(part 1 of 3)
# Autodesk Inventor assembly: FinalAssembly
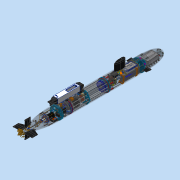
[picture p0: Inventor's stored thumbnail of the model, 180x180]
Saved by Autodesk Inventor 2018 (Build 220112000, 112)
## iProperties
Created: 2016-12-11
Part Number: FinalAssembly
Document SubType Name: Assembly
Designer: techn
Mass: 4957.63 g
Surface Area: 18369.4 cm^2
Volume: 2887.61 cm^3
Density: 1.71686 g/cm^3
Author: techn
## Documents named in this file (168)
- D:\Projects\Submarine-project\CAD\FinalAssembly.iam
- D:\Projects\Submarine-project\CAD\aft\AftSectionAirtightRear.ipt
- D:\Projects\Submarine-project\CAD\aft\AftSectionWithSteeringLinkages.ipt
- D:\Projects\Submarine-project\CAD\aft\RearmostAftSection.ipt
- D:\Projects\Submarine-project\CAD\common\steeringYoke3mmShaft.ipt
- D:\Projects\Submarine-project\CAD\aft\aftSectionAirtightCap.ipt
- D:\Projects\Submarine-project\CAD\common\AluminumSealingDisc.ipt
- D:\Projects\Submarine-project\CAD\midships\AftServoSection\rearServoAttachmentPlate.ipt
- D:\Projects\Submarine-project\CAD\common\HitecServo\HitecServoAssembly.iam
- D:\Projects\Submarine-project\CAD\common\HitecServo\ServoHorn10mmPitch.ipt
- D:\Projects\Submarine-project\CAD\aft\planeLinkages\2mmBentFromSealDive.ipt
- D:\Projects\Submarine-project\CAD\aft\planeLinkages\2mmToDive.ipt
- D:\Projects\Submarine-project\CAD\aft\planeLinkages\2mmToSeal.ipt
- D:\Projects\Submarine-project\CAD\aft\planeLinkages\2mmToServo.ipt
- D:\Projects\Submarine-project\CAD\aft\planeLinkages\metalClevisis.ipt
- D:\Projects\Submarine-project\CAD\aft\planeLinkages\2mmBentFromSealRudder.ipt
- D:\Projects\Submarine-project\CAD\aft\planeLinkages\2mmToRudder.ipt
- D:\Projects\Submarine-project\CAD\common\screws\flatPlasticScrewSmall.ipt
- D:\Projects\Submarine-project\CAD\common\YokeDowelPins.ipt
- D:\Projects\Submarine-project\CAD\aft\RudderStabilizingLowerFins.ipt
- D:\Projects\Submarine-project\CAD\common\SleeveBearing3mmFlanged.ipt
- D:\Projects\Submarine-project\CAD\aft\DivePlanesStabilizingFins.ipt
- D:\Projects\Submarine-project\CAD\aft\RudderStabilizingFinBottom.ipt
- D:\Projects\Submarine-project\CAD\aft\RudderStabilizingFins.ipt
- D:\Projects\Submarine-project\CAD\aft\3mmControlSurfaceShaft_1.ipt
- D:\Projects\Submarine-project\CAD\aft\3mmControlSurfaceShaft_2.ipt
- D:\Projects\Submarine-project\CAD\aft\DivePlanesControlSurface.ipt
- D:\Projects\Submarine-project\CAD\aft\RudderLowerControlSurface.ipt
- D:\Projects\Submarine-project\CAD\aft\RudderUpperControlSurface.ipt
- D:\Projects\Submarine-project\CAD\common\screws\ScrewPlastic_4_20_.625inch.ipt
- D:\Projects\Submarine-project\CAD\common\ThreadedRod_Nuts_Bolts\NarrowHexNutThread_5_40.ipt
- D:\Projects\Submarine-project\CAD\common\ORingA50_.25OD_.125ID.ipt
- D:\Projects\Submarine-project\CAD\common\ThreadedRod_Nuts_Bolts\Bolt_ButtonHead_Hex_Thread_5_40_1inch.ipt
- D:\Projects\Submarine-project\CAD\aft\MotorAssembly0.iam
- D:\Projects\Submarine-project\CAD\common\PushRodSeal\Engel3mm\Engel3mmAssembly.iam
- D:\Projects\Submarine-project\CAD\common\ThreadedRod_Nuts_Bolts\Bolt_Buttonhead_Hex_Thread_5_40_.625inch.ipt
- D:\Projects\Submarine-project\CAD\common\ORingA50_1.296ID_1.574OD.ipt
- D:\Projects\Submarine-project\CAD\midships\ElectronicsSection\QUICRUN ESC\QuicrunESCAssembly.iam
- D:\Projects\Submarine-project\CAD\common\screws\ScrewPlastic_4_20_.75inch_Flat.ipt
- D:\Projects\Submarine-project\CAD\common\ThreadedRod_Nuts_Bolts\Bolt_FlatHead_Hex_Thread_M3_8mm.ipt
- D:\Projects\Submarine-project\CAD\common\ORingA50_3.75OD_3.5ID_Compressed.ipt
- D:\Projects\Submarine-project\CAD\midships\AftServoSection\frontServoAttachmentPlate.ipt
- D:\Projects\Submarine-project\CAD\midships\AluminumSealingDiscMidshipsRear.ipt
- D:\Projects\Submarine-project\CAD\midships\SpoolSection\aftSpoolSectionSealingWall.ipt
- D:\Projects\Submarine-project\CAD\common\3mmShaftToServo\ServoWithShaftAssembly.iam
- D:\Projects\Submarine-project\CAD\common\screws\ScrewPlastic_4_20_.5inch.ipt
- D:\Projects\Submarine-project\CAD\common\ORingA70_.176ID_.316OD.ipt
- D:\Projects\Submarine-project\CAD\midships\ElectronicsSection\aluminumWiringTubing.ipt
- D:\Projects\Submarine-project\CAD\common\ThreadedRod_Nuts_Bolts\aftThreadedRodThread_5_40.ipt
- D:\Projects\Submarine-project\CAD\common\SleeveBearing.125inch.ipt
- D:\Projects\Submarine-project\CAD\common\BallBearing4mmFlanged.ipt
- D:\Projects\Submarine-project\CAD\midships\BallastSection\bearing_1_8inch.ipt
- D:\Projects\Submarine-project\CAD\midships\SpoolSection\PinionGear.ipt
- D:\Projects\Submarine-project\CAD\midships\SpoolSection\SpoolAxle.ipt
- D:\Projects\Submarine-project\CAD\midships\BallastSection\smallIdlerPinion.ipt
- D:\Projects\Submarine-project\CAD\midships\SpoolSection\SpoolSectionSealingWallFront.ipt
- D:\Projects\Submarine-project\CAD\midships\SpoolSection\FixedCylinderWireStorage.ipt
- D:\Projects\Submarine-project\CAD\midships\SpoolSection\FixedCylinderWireStorageInsert.ipt
- D:\Projects\Submarine-project\CAD\midships\BallastSection\pistonTank.ipt
- D:\Projects\Submarine-project\CAD\common\SleeveBearing3mm.ipt
- D:\Projects\Submarine-project\CAD\midships\BallastSection\pistonSealingWallFront.ipt
- D:\Projects\Submarine-project\CAD\midships\BallastSection\pistonSealingDisc.ipt
- D:\Projects\Submarine-project\CAD\midships\BallastSection\pistonSealingWallRear.ipt
- D:\Projects\Submarine-project\CAD\common\ThreadedRod_Nuts_Bolts\WeldNutThread_5_16_18.ipt
- D:\Projects\Submarine-project\CAD\common\ThreadedRod_Nuts_Bolts\ThreadedRodThread_5_16_18.ipt
- D:\Projects\Submarine-project\CAD\common\ThreadedRod_Nuts_Bolts\HexNutThread_5_16_18.ipt
- D:\Projects\Submarine-project\CAD\common\ThreadedRod_Nuts_Bolts\WasherForThread_5_16_18.ipt
- D:\Projects\Submarine-project\CAD\midships\BallastSection\forwardBallastSealingWallRear.ipt
- D:\Projects\Submarine-project\CAD\midships\BallastSection\forwardBallastSealingWallFront.ipt
- D:\Projects\Submarine-project\CAD\midships\BallastSection\forwardBallastSealingWallDisc.ipt
- D:\Projects\Submarine-project\CAD\common\ThreadedRod_Nuts_Bolts\midshipsThreadedRodThread_5_40.ipt
- D:\Projects\Submarine-project\CAD\midships\BallastSection\pushSwitchBushingHolder.ipt
- D:\Projects\Submarine-project\CAD\midships\BallastSection\pushSwitchRod.ipt
- D:\Projects\Submarine-project\CAD\midships\BallastSection\pushSwitchSpring.ipt
- D:\Projects\Submarine-project\CAD\midships\BallastSection\RadialBearingMountCover.ipt
- D:\Projects\Submarine-project\CAD\midships\BallastSection\ThrustWasher.ipt
- D:\Projects\Submarine-project\CAD\midships\BallastSection\pistonSpurGear.ipt
- D:\Projects\Submarine-project\CAD\midships\BallastSection\retentionStandoffs.ipt
- D:\Projects\Submarine-project\CAD\midships\BallastSection\SpurGearThrustDistributer.ipt
- D:\Projects\Submarine-project\CAD\midships\BallastSection\ThrustBearingMount.ipt
- D:\Projects\Submarine-project\CAD\midships\BallastSection\idlerShaftBearingMount.ipt
- D:\Projects\Submarine-project\CAD\aft\540DCMotor.ipt
- D:\Projects\Submarine-project\CAD\midships\BallastSection\limitSwitchPushHolder1.ipt
- D:\Projects\Submarine-project\CAD\common\ThreadedRod_Nuts_Bolts\WeldNutThread_5_16_18_Cut.ipt
- D:\Projects\Submarine-project\CAD\midships\BallastSection\limitSwitchHolder2Backplate.ipt
- D:\Projects\Submarine-project\CAD\common\Switches\LimitSwitch\LIMIT SWITCH.ipt
- D:\Projects\Submarine-project\CAD\midships\BallastSection\limitSwitchHolderMount.ipt
- D:\Projects\Submarine-project\CAD\midships\BallastSection\limitSwitchHolder2.ipt
- D:\Projects\Submarine-project\CAD\common\Switches\LimitSwitch\LimitSwitchAssembly.iam
- D:\Projects\Submarine-project\CAD\midships\BallastSection\idlerShaft.ipt
- D:\Projects\Submarine-project\CAD\midships\BallastSection\largeIdlerPinion.ipt
- D:\Projects\Submarine-project\CAD\midships\BallastSection\BearingRetentionBrace.ipt
- D:\Projects\Submarine-project\CAD\midships\ElectronicsSection\foreElectronicsSealingWallRear.ipt
- D:\Projects\Submarine-project\CAD\midships\ElectronicsSection\foreElectronicsSealingDisc.ipt
- D:\Projects\Submarine-project\CAD\midships\ElectronicsSection\foreElectronicsSealingWallFront.ipt
- D:\Projects\Submarine-project\CAD\midships\ElectronicsSection\foreElectronicsSealingWallFrontCap.ipt
- D:\Projects\Submarine-project\CAD\midships\3mmControlSurfaceShaftForePlanes.ipt
- D:\Projects\Submarine-project\CAD\midships\foreDivePlanes.ipt
- D:\Projects\Submarine-project\CAD\midships\foreDivePlanesLinkage.ipt
- D:\Projects\Submarine-project\CAD\fore\foreHullLower.ipt
- D:\Projects\Submarine-project\CAD\fore\foreHullInsert.ipt
- D:\Projects\Submarine-project\CAD\fore\foreHullUpper.ipt
- D:\Projects\Submarine-project\CAD\midships\ElectronicsSection\ArduinoMegaHolder1.ipt
- D:\Projects\Submarine-project\CAD\midships\ElectronicsSection\ArduinoMegaHolder2.ipt
- D:\Projects\Submarine-project\CAD\midships\ElectronicsSection\ArduinoMega.ipt
- D:\Projects\Submarine-project\CAD\midships\ElectronicsSection\ServoControllerHolder.ipt
- D:\Projects\Submarine-project\CAD\midships\ElectronicsSection\ServoController\ServoControllerAssembly.iam
- D:\Projects\Submarine-project\CAD\midships\ElectronicsSection\ArduinoNanoHolder.ipt
- D:\Projects\Submarine-project\CAD\midships\ElectronicsSection\ArduinoNanoHolderSide2.ipt
- D:\Projects\Submarine-project\CAD\midships\ElectronicsSection\ArduinoNanoNoPins.iam
- D:\Projects\Submarine-project\CAD\midships\ElectronicsSection\BEC\BEC_Assembly.iam
- D:\Projects\Submarine-project\CAD\midships\PrimaryHullLexanTube_01.ipt
- D:\Projects\Submarine-project\CAD\common\5mmLED.ipt
- D:\Projects\Submarine-project\CAD\ASDS\ASDSAssembly.iam
- D:\Projects\Submarine-project\CAD\common\DriveBattery.ipt
- D:\Projects\Submarine-project\CAD\common\DriveBatteryHolder.ipt
- D:\Projects\Submarine-project\CAD\common\ElectronicsBatteryAssembly.iam
- D:\Projects\Submarine-project\CAD\common\PressureSensor.ipt
- D:\Projects\Submarine-project\CAD\midships\Sail\SailAssembly\SailAssembly.iam
- D:\Projects\Submarine-project\CAD\midships\ElectronicsSection\BackupNanoCase.iam
- D:\Projects\Submarine-project\CAD\common\RelayModule.ipt
- D:\Projects\Submarine-project\CAD\midships\Sail\WireGuide.ipt
- D:\Projects\Submarine-project\CAD\midships\Sail\WireGuideToSail1.ipt
- D:\Projects\Submarine-project\CAD\midships\Sail\WireGuideToSail2.ipt
- D:\Projects\Submarine-project\CAD\midships\Sail\WireGuideToMiniSub.ipt
- D:\Projects\Submarine-project\CAD\midships\Sail\WireGuideToMiniSubExtender.ipt
- D:\Projects\Submarine-project\CAD\midships\SpoolSection\SmallSpoolAssembly.iam
- D:\Projects\Submarine-project\CAD\midships\SpoolSection\CarriageImproved.ipt
- D:\Projects\Submarine-project\CAD\midships\AftServoSection\MiniSpoolServoShaft.ipt
- D:\Projects\Submarine-project\CAD\midships\AftServoSection\CarriageConnectorShaft.ipt
- D:\Projects\Submarine-project\CAD\midships\SpoolSection\carriageRideShaft.ipt
- D:\Projects\Submarine-project\CAD\common\ThreadedRod_Nuts_Bolts\spoolCarriageThreadedRodThread_5_40.ipt
- D:\Projects\Submarine-project\CAD\common\ThreadedRod_Nuts_Bolts\aftServoSectionThreadedRodThread_5_40.ipt
- D:\Projects\Submarine-project\CAD\common\PinionGear20T.ipt
- D:\Projects\Submarine-project\CAD\midships\SpoolSection\CarrageRodEndMount.ipt
- D:\Projects\Submarine-project\CAD\midships\AftServoSection\SpoolServoMount.ipt
- D:\Projects\Submarine-project\CAD\common\ORingA70_2.484ID_2.762OD_Compressed.ipt
- D:\Projects\Submarine-project\CAD\common\NarrowHexNutCaps.ipt
- D:\Projects\Submarine-project\CAD\aft\encoder\4mmShaftCollar.ipt
- D:\Projects\Submarine-project\CAD\aft\encoder\ShaftCollarMagnetMount.ipt
- D:\Projects\Submarine-project\CAD\aft\encoder\EncoderMagnet.ipt
- D:\Projects\Submarine-project\CAD\midships\BallastSection\idlerShaft2.ipt
- D:\Projects\Submarine-project\CAD\common\ThreadedRod_Nuts_Bolts\Bolt_SocketHead_Hex_Thread_M3_16mm.ipt
- D:\Projects\Submarine-project\CAD\midships\BallastSection\CompressionWasherPlastic.ipt
- D:\Projects\Submarine-project\CAD\common\ThreadedRod_Nuts_Bolts\HexNutThread_M3.ipt
- D:\Projects\Submarine-project\CAD\midships\BallastSection\ThrustWasherPrimary.ipt
- D:\Projects\Submarine-project\CAD\midships\BallastSection\pushSwitchRodSpacer.ipt
- D:\Projects\Submarine-project\CAD\midships\BallastSection\RadialBearingLarge.ipt
- D:\Projects\Submarine-project\CAD\Downloaded\ScimitarProp\ScimitarPropellerModel1.iam
- D:\Projects\Submarine-project\CAD\common\MicroGearMotor\MicroGearMotor.ipt
- D:\Projects\Submarine-project\CAD\common\3mm_.125inch_ShaftCoupler.ipt
- D:\Projects\Submarine-project\CAD\common\MicroGearMotor\GearMotorMount.ipt
- D:\Projects\Submarine-project\CAD\midships\ASDSAttachment\ASDSAttachmentAssemblyUpdated.iam
- D:\Projects\Submarine-project\CAD\midships\ASDSAttachment\RearMount.ipt
- D:\Projects\Submarine-project\CAD\aft\encoder\hallEffectSensorAssembly.iam
- D:\Projects\Submarine-project\CAD\midships\BallastSection\gearboxBearingHolderForward.ipt
- D:\Projects\Submarine-project\CAD\midships\BallastSection\gearboxBearingHolderHexNutBacking.ipt
- D:\Projects\Submarine-project\CAD\common\ThreadedRod_Nuts_Bolts\Bolt_SocketHead_Hex_Thread_M3_8mm.ipt
- D:\Projects\Submarine-project\CAD\common\ThreadedRod_Nuts_Bolts\Bolt_ButtonHead_Hex_Thread_M3_10mm.ipt
- D:\Projects\Submarine-project\CAD\common\MicroGearMotor\GearMotorMountArm.ipt
- D:\Projects\Submarine-project\CAD\midships\AftServoSection\HallEffectSpoolSensorMount2.ipt
- D:\Projects\Submarine-project\CAD\aft\encoder\HallEffectSensor.ipt
- D:\Projects\Submarine-project\CAD\midships\AftServoSection\SpoolCarrageMagnetMountREV2.ipt
- D:\Projects\Submarine-project\CAD\midships\AftServoSection\HallEffectSpoolSensorMount3.ipt
- D:\Projects\Submarine-project\CAD\midships\AftServoSection\HallEffectSpoolSensorMount3Brace.ipt
- D:\Projects\Submarine-project\CAD\midships\BallastSection\HallEffectSpoolSensorMount3.ipt
- D:\Projects\Submarine-project\CAD\midships\ElectronicsSection\RelayHolderREV2.ipt
- D:\Projects\Submarine-project\CAD\SlipRing\SlipRingAssy.iam
## Components (560 placed, 166 different names)
1. AftSectionAirtightRear:1 — Mate:1, Mate:5, Mate:6, Mate:101, Mate:205, Angle:13, Mate:221, Mate:223, Mate:224, Mate:225, Angle:15, Mate:226, Mate:227, Angle:16, Rigid:11, Mate:228, Mate:229, Rigid:12, Flush:16, Flush:54, Flush:55, Mate:428, Mate:436, Mate:437, Mate:441, Mate:700
2. AftSectionWithSteeringLinkages:1 — Mate:1, Mate:30, Mate:31, Mate:190, Angle:11, Mate:436, Mate:1031, Rigid:38, Rigid:39, Mate:1061, Mate:1062, Mate:1063, Mate:1064, Mate:1065
3. AluminumSealingDisc:1 — Mate:8, Mate:10, Mate:11, Mate:12, Mate:13, Mate:102, Rigid:13
4. rearServoAttachmentPlate:1 — Mate:11, Mate:12, Mate:13, Mate:14, Mate:16, Mate:17, Mate:18, Mate:19, Mate:249, Mate:261, Mate:275, Mate:427, Mate:858
5. HitecServoAssembly:1 [sub-assembly] — Mate:14, Mate:16, Mate:20, Mate:23, Angle:5, Flush:17, Mate:293, Mate:296, Mate:297, Angle:26, Mate:427, Angle:82
6. HitecServoAssembly:2 [sub-assembly] — Mate:17, Mate:18, Mate:19, Mate:21, Mate:22, Angle:4, Angle:18, Angle:70, Angle:84
7. ServoHorn10mmPitch:1 — Mate:20, Mate:23, Mate:37, Angle:5
8. ServoHorn10mmPitch:2 — Mate:21, Mate:22, Mate:36, Angle:4
9. aftSectionAirtightCap:2 — Mate:5, Mate:6, Mate:8, Mate:10, Mate:101, Mate:102, Mate:219, Mate:220, Angle:14, Mate:244, Flush:18, Mate:701
10. RearmostAftSection:2 — Mate:28, Mate:29, Mate:30, Mate:31, Mate:109, Mate:110, Mate:111, Mate:112, Mate:113, Mate:114, Mate:118, Mate:119, Mate:120, Mate:121, Mate:122, Mate:123, Mate:124, Mate:125, Mate:126, Mate:127, Mate:128, Mate:129, Mate:130, Mate:131, Mate:132, Mate:133, Mate:134, Mate:135, Mate:136, Angle:6, Mate:137, Mate:138, Angle:7, Mate:160, Mate:161, Mate:162, Mate:163, Mate:164, Mate:165, Mate:166, Mate:167, Mate:168, Mate:169, Mate:170, Mate:171, Mate:206, Mate:216, Mate:313, Mate:314, Mate:438, Mate:439, Mate:440
11. BallBearing4mmFlanged:1 — Mate:313, Mate:314, Mate:1030
12. steeringYoke3mmShaft:3 — Mate:29, Mate:59, Mate:60, Flush:8, Flush:9, Rigid:1
13. steeringYoke3mmShaft:4 — Mate:28, Mate:61, Mate:77, Rigid:2
14. metalClevisis:5 — Mate:36, Mate:71, Mate:72, Mate:707, Flush:113
15. metalClevisis:6 — Mate:37, Mate:55, Mate:56, Mate:706, Flush:112
16. 2mmToServo:7 — Mate:55, Mate:56, Ball:3
17. 2mmToSeal:4 — Ball:2
18. 2mmToSeal:5 — Ball:3
19. 2mmToDive:1 — Ball:1
20. metalClevisis:7 — Mate:59, Mate:60, Mate:69, Mate:70, Flush:7, Mate:430
21. metalClevisis:8 — Mate:61, Mate:75, Mate:76, Mate:77, Flush:6, Mate:429
22. 2mmBentFromSealDive:2 — Ball:1, Mate:69, Mate:70
23. 2mmToServo:8 — Ball:2, Mate:71, Mate:72
24. 2mmToRudder:1 — Ball:4
25. 2mmBentFromSealRudder:2 — Ball:4, Mate:75, Mate:76
26. YokeDowelPins:1 — Flush:6, Mate:429
27. YokeDowelPins:2 — Flush:7, Mate:430
28. RudderStabilizingLowerFins:1 — Mate:109, Mate:110, Mate:111
29. RudderStabilizingLowerFins:2 — Mate:112, Mate:113, Mate:114, Mate:158
30. RudderStabilizingLowerFins:3 — Mate:438, Mate:439, Mate:440
31. RudderStabilizingLowerFins:4 — Mate:118, Mate:119, Mate:120
32. SleeveBearing3mmFlanged:1 — Mate:121, Mate:122, Mate:141
33. SleeveBearing3mmFlanged:2 — Mate:127, Mate:128, Mate:139
34. SleeveBearing3mmFlanged:3 — Mate:125, Mate:126, Mate:142
35. SleeveBearing3mmFlanged:4 — Mate:123, Mate:124, Mate:140
36. DivePlanesStabilizingFins:1 — Mate:129, Mate:133, Mate:134
37. DivePlanesStabilizingFins:2 — Mate:130, Mate:131, Mate:132, Mate:148
38. RudderStabilizingFinBottom:1 — Mate:137, Mate:138, Angle:7
39. RudderStabilizingFins:1 — Mate:135, Mate:136, Angle:6
40. 3mmControlSurfaceShaft_1:1 — Mate:139, Mate:143, Mate:144, Flush:9, Rigid:1
41. 3mmControlSurfaceShaft_1:2 — Mate:140, Mate:147, Mate:150, Flush:8
42. 3mmControlSurfaceShaft_2:1 — Mate:141, Mate:153, Mate:154, Rigid:2
43. 3mmControlSurfaceShaft_2:2 — Mate:142, Mate:155, Mate:156
44. DivePlanesControlSurface:1 — Mate:143, Mate:144, Mate:149
45. DivePlanesControlSurface:2 — Mate:147, Mate:148, Mate:149, Mate:150
46. YokeDowelPins:3 — Mate:707, Flush:113
47. YokeDowelPins:4 — Mate:706, Flush:112
48. RudderLowerControlSurface:1 — Mate:155, Mate:156, Mate:158, Mate:159
49. RudderUpperControlSurface:1 — Mate:153, Mate:154, Mate:159
50. ScrewPlastic_4_20_.625inch:1 — Mate:160, Mate:161
51. ScrewPlastic_4_20_.625inch:2 — Mate:162, Mate:163
52. ScrewPlastic_4_20_.625inch:3 — Mate:166, Mate:167
53. ScrewPlastic_4_20_.625inch:6 — Mate:170, Mate:171
54. ScrewPlastic_4_20_.625inch:7 — Mate:164, Mate:165
55. ScrewPlastic_4_20_.625inch:8 — Mate:168, Mate:169
56. MotorAssembly0:1 [sub-assembly] — Mate:221, Mate:223, Mate:231, Tangent:1, Mate:259, Mate:260, Flush:20, Flush:21, Mate:441, Mate:921, Mate:1029
57. Engel3mmAssembly:1 [sub-assembly] — Mate:226, Mate:227, Angle:16, Angle:17
58. Engel3mmAssembly:2 [sub-assembly] — Mate:224, Mate:225, Angle:15
59. ORingA50_1.296ID_1.574OD:1 — Rigid:12
60. QuicrunESCAssembly:1 [sub-assembly] — Tangent:1, Angle:18, Flush:16, Flush:17, Angle:61
61. Bolt_FlatHead_Hex_Thread_M3_8mm:1 — Mate:260, Flush:20
62. Bolt_FlatHead_Hex_Thread_M3_8mm:2 — Mate:259, Flush:21
63. ORingA50_3.75OD_3.5ID_Compressed:1 — Rigid:13
64. frontServoAttachmentPlate:1 — Mate:261, Mate:269, Mate:270, Mate:271, Mate:274, Mate:293, Mate:301, Mate:302, Mate:830, Mate:831, Mate:836, Mate:839, Mate:840, Flush:122, Mate:860, Rigid:35, Mate:1114, Mate:1128
65. AluminumSealingDiscMidshipsRear:1 — Mate:269, Mate:270, Mate:271, Mate:272, Mate:273, Rigid:17, Rigid:28, Mate:846, Mate:848, Rigid:31, Rigid:32, Mate:889
66. aftSpoolSectionSealingWall:1 — Mate:272, Mate:273, Mate:274, Mate:300, Mate:305, Mate:335, Mate:336, Mate:373, Mate:827, Mate:828, Mate:829, Mate:837, Mate:838, Mate:845, Mate:847, Mate:849, Flush:124, Mate:865, Mate:866, Flush:127, Rigid:36
67. ORingA50_3.75OD_3.5ID_Compressed:2 — Rigid:32
68. ServoWithShaftAssembly:1 [sub-assembly] — Mate:713, Mate:889, Angle:61, Mate:892, Mate:893, Mate:894, Mate:895, Mate:896, Flush:130, Angle:79, Flush:502, Angle:80
69. PinionGear:1 — Mate:713, Flush:120, Flush:130
70. SpoolAxle:1 — Mate:335, Mate:336, Mate:377, Mate:383, Mate:826
71. SpoolSectionSealingWallFront:1 — Mate:373, Mate:374, Mate:379, Mate:380, Mate:385, Flush:52, Mate:387, Mate:388, Mate:390, Mate:1148
72. FixedCylinderWireStorage:1 — Mate:377, Mate:379, Mate:380, Mate:384, Angle:24, Flush:74, Mate:1147
73. FixedCylinderWireStorageInsert:1 — Mate:383, Mate:384, Angle:24, Mate:526
74. pistonTank:1 — Mate:388, Mate:390, Mate:396, Mate:397, Mate:399, Mate:418, Mate:419, Angle:37
75. pistonSealingWallFront:1 — Mate:396, Mate:402, Mate:410, Rigid:20, Mate:414, Mate:415, Angle:86
76. pistonSealingDisc:1 — Mate:397, Mate:401, Mate:402, Rigid:33, Rigid:34
77. pistonSealingWallRear:1 — Mate:399, Mate:401, Mate:405, Mate:407, Mate:417, Mate:914, Flush:132, Angle:85
78. WeldNutThread_5_16_18:1 — Mate:406, Mate:407, Mate:412, Mate:413, Angle:26
79. ThreadedRodThread_5_16_18:1 — Mate:405, Mate:406, Mate:408, Mate:409, Flush:53, Mate:478, Mate:505, Flush:67, Mate:1005, Rotation/Translation:1
80. HexNutThread_5_16_18:1 — Mate:408, Mate:411, Flush:53
81. WasherForThread_5_16_18:1 — Mate:409, Mate:410, Mate:411
82. forwardBallastSealingWallRear:1 — Mate:418, Mate:419, Mate:420, Mate:421, Mate:423
83. forwardBallastSealingWallFront:1 — Mate:424, Mate:425, Mate:426, Mate:444, Mate:445, Angle:28, Mate:446, Mate:447, Mate:451, Mate:452, Mate:453, Mate:461, Mate:463, Mate:464, Mate:465, Mate:466, Mate:476, Mate:481, Mate:585, Flush:149, Flush:153, Rigid:37, Angle:73, Mate:1072, Mate:1074, Mate:1075, Mate:1076, Flush:499, Flush:500, Mate:1089, Mate:1090, Mate:1092, Mate:1093, Mate:1096, Mate:1097, Mate:1099
84. forwardBallastSealingWallDisc:1 — Mate:421, Mate:422, Mate:423, Mate:424, Mate:426, Rigid:21, Rigid:23, Mate:1021
85. ORingA50_3.75OD_3.5ID_Compressed:3 — Rigid:21
86. pushSwitchBushingHolder:1 — Mate:447, Mate:451, Flush:57, Flush:58
87. flatPlasticScrewSmall:19 — Mate:452, Flush:57
88. flatPlasticScrewSmall:20 — Mate:453, Flush:58
89. RadialBearingLarge:1
90. pushSwitchRod:1 — Mate:456, Mate:1022, Mate:1025, Mate:1099
91. pushSwitchSpring:1 — Mate:456, Mate:1023
92. WeldNutThread_5_16_18:2 — Mate:1008, Angle:63, Angle:64, Mate:1100, Mate:1101
93. RadialBearingMountCover:1 — Mate:463, Mate:464, Mate:465, Flush:61, Mate:469, Mate:470
94. ThrustWasher:1 — Mate:469, Mate:470, Mate:1006, Mate:1007
95. SpurGearThrustDistributer:1 — Mate:478, Mate:1013, Angle:65
96. ThrustBearingMount:1 — Mate:480, Mate:481, Mate:482, Mate:486, Mate:488, Flush:490, Mate:499, Mate:500, Mate:501, Mate:513, Mate:514, Mate:515, Mate:516, Mate:517, Mate:734, Mate:965, Flush:146, Mate:966, Flush:147, Mate:967, Flush:148, Mate:968, Mate:969, Mate:970, Mate:974, Mate:975, Mate:976, Mate:992, Mate:999, Mate:1000, Mate:1001, Mate:1002, Mate:1003, Mate:1004, Mate:1014, Mate:1015, Mate:1023, Mate:1024, Mate:1027, Mate:1135, Mate:1136
97. SleeveBearing.125inch:7 — Mate:488, Flush:490
98. limitSwitchPushHolder1:1 — Mate:499, Mate:500, Mate:501, Mate:502, Mate:503, Mate:504, Flush:64, Flush:65, Flush:66, Mate:506, Mate:507, Angle:35, Mate:508, Mate:509, Mate:510, Mate:511, Mate:512, Mate:698, Flush:109
99. flatPlasticScrewSmall:27 — Mate:502, Flush:64
100. flatPlasticScrewSmall:28 — Mate:503, Flush:66
101. flatPlasticScrewSmall:29 — Mate:504, Flush:65
102. WeldNutThread_5_16_18_Cut:1 — Mate:505, Flush:67, Angle:34
103. limitSwitchHolder2Backplate:1 — Mate:506, Mate:507, Angle:35, Flush:68, Flush:69
104. flatPlasticScrewSmall:30 — Mate:508, Flush:68
105. LIMIT SWITCH:1 — Mate:509, Mate:510, Mate:511
106. flatPlasticScrewSmall:31 — Mate:512, Flush:69
107. limitSwitchHolderMount:1 — Mate:513, Mate:514, Mate:515, Flush:70, Flush:71, Mate:518, Mate:519, Mate:520, Mate:521, Mate:522
108. flatPlasticScrewSmall:32 — Mate:516, Flush:70
109. flatPlasticScrewSmall:33 — Mate:517, Flush:71
110. limitSwitchHolder2:1 — Mate:518, Mate:519, Mate:520, Flush:72, Flush:73, Mate:523, Mate:524, Mate:525, Angle:87
111. flatPlasticScrewSmall:34 — Mate:521, Flush:72
112. flatPlasticScrewSmall:35 — Mate:522, Flush:73
113. LimitSwitchAssembly:1 [sub-assembly] — Mate:523, Mate:524, Mate:525
114. foreElectronicsSealingWallRear:1 — Mate:585, Mate:586, Mate:587, Mate:588, Mate:591, Mate:596, Mate:597, Mate:598, Angle:38, Mate:685
115. foreElectronicsSealingDisc:1 — Mate:587, Mate:588, Mate:589, Mate:590, Rigid:25
116. foreElectronicsSealingWallFront:1 — Mate:590, Mate:591, Mate:592, Flush:91, Rigid:24, Mate:594, Mate:601, Flush:92, Flush:93, Mate:611, Mate:612, Mate:613, Mate:614, Mate:615, Mate:616, Angle:39, Mate:617, Mate:618, Angle:40, Tangent:2, Tangent:3, Mate:626, Mate:631, Mate:632, Angle:42, Mate:633, Mate:634, Mate:635, Mate:642, Mate:738
117. ORingA50_3.75OD_3.5ID_Compressed:4 — Rigid:25
118. HitecServoAssembly:3 [sub-assembly] — Mate:597, Mate:598, Angle:38, Mate:599, Mate:600, Mate:627, Mate:628, Angle:45, Flush:108, Angle:53, Flush:118, Angle:54
119. foreElectronicsSealingWallFrontCap:1 — Mate:601, Flush:92, Flush:93, Angle:49
120. SleeveBearing3mm:4 — Mate:611, Mate:612, Mate:623
121. SleeveBearing3mm:5 — Mate:613, Mate:614, Mate:624
122. Engel3mmAssembly:5 [sub-assembly] — Mate:615, Mate:616, Angle:39
123. Engel3mmAssembly:6 [sub-assembly] — Mate:617, Mate:618, Angle:40
124. 3mmControlSurfaceShaftForePlanes:1 — Mate:619, Mate:620, Mate:623
125. 3mmControlSurfaceShaftForePlanes:2 — Mate:621, Mate:622, Mate:624, Mate:625
126. foreDivePlanes:1 — Mate:619, Mate:620, Tangent:3, Flush:103
127. foreDivePlanes:2 — Mate:621, Mate:622, Tangent:2, Flush:103, Angle:41
128. steeringYoke3mmShaft:5 — Mate:625, Mate:626, Angle:41, Mate:630
129. ServoHorn10mmPitch:3 — Mate:627, Mate:628, Mate:629, Tangent:4
130. foreDivePlanesLinkage:2 — Mate:629, Mate:630, Tangent:4
131. foreHullLower:1 — Mate:633, Mate:634, Mate:635, Mate:636, Mate:637, Mate:641
132. foreHullInsert:1 — Mate:638, Mate:639, Mate:640, Mate:642, Mate:643, Flush:104, Flush:110
133. foreHullUpper:1 — Mate:638, Mate:639, Mate:640, Mate:641, Angle:43, Mate:702, Mate:703
134. ArduinoMegaHolder1:1 — Mate:644, Mate:645, Mate:648, Mate:650, Mate:685, Mate:691, Mate:689
135. ArduinoMegaHolder2:1 — Mate:646, Mate:647, Mate:649, Mate:651, Mate:686, Mate:687, Mate:693, Mate:695
136. ArduinoMega:1 — Mate:648, Mate:649, Mate:650, Mate:651, Angle:44
137. ServoControllerHolder:1 — Mate:654, Mate:655, Mate:656, Mate:657, Mate:658, Mate:659, Mate:660, Mate:663
138. ServoControllerHolder:2 — Mate:654, Mate:656, Mate:661, Mate:687, Mate:995
139. ServoControllerAssembly:1 [sub-assembly] — Mate:658, Mate:659, Mate:660, Mate:661
140. ArduinoNanoHolder:1 — Mate:666, Mate:667, Mate:668, Flush:105, Flush:106, Mate:682, Mate:1140, Angle:88, Mate:1142, Angle:89
141. ArduinoNanoHolderSide2:1 — Mate:664, Mate:665, Mate:668, Mate:672, Mate:674, Mate:676, Mate:686
142. ArduinoNanoNoPins:1 [sub-assembly] — Mate:672, Flush:105, Flush:106
143. NarrowHexNutThread_5_40:147 — Mate:673, Mate:674
144. NarrowHexNutThread_5_40:148 — Mate:675, Mate:676
145. NarrowHexNutThread_5_40:151 — Mate:681, Mate:682
146. NarrowHexNutThread_5_40:168 — Mate:692, Mate:693
147. NarrowHexNutThread_5_40:169 — Mate:694, Mate:695
148. QuicrunESCAssembly:2 [sub-assembly] — Tangent:5, Angle:44, Angle:45, Mate:698, Flush:108
149. BEC_Assembly:1 [sub-assembly] — Tangent:6, Flush:109, Mate:734
150. PrimaryHullLexanTube_01:1 — Mate:700, Mate:701, Angle:46, Mate:736, Mate:737, Mate:802, Mate:803, Mate:804, Mate:813, Mate:817, Mate:820, Mate:1059, Mate:1060
151. 5mmLED:1 — Mate:702, Flush:110, Flush:111
152. 5mmLED:2 — Mate:703, Flush:111
153. ASDSAssembly:1 [sub-assembly]
154. DriveBattery:2 — Mate:721, Mate:722, Mate:723, Mate:724, Flush:116
155. DriveBatteryHolder:1 — Mate:721, Mate:724, Mate:725, Flush:116
156. DriveBatteryHolder:2 — Mate:722, Mate:723, Mate:725, Mate:726, Mate:727
157. ElectronicsBatteryAssembly:1 [sub-assembly] — Angle:49, Flush:117
158. SailAssembly:1 [sub-assembly] — Mate:736, Angle:52, Mate:737, Mate:805, Mate:807, Mate:808, Mate:812, Mate:814, Mate:816
159. PressureSensor:2 — Mate:738, Angle:53, Mate:739, Flush:118
160. BackupNanoCase:1 [sub-assembly] — Mate:780, Angle:54
161. WireGuide:1 — Mate:802, Mate:806, Mate:808
162. WireGuide:2 — Mate:803, Mate:812, Mate:815, Mate:818
163. WireGuideToSail1:1 — Mate:804, Mate:805, Mate:806, Mate:807
164. WireGuideToSail2:1 — Mate:813, Mate:814, Mate:815, Mate:816, Mate:819
165. WireGuideToMiniSub:1 — Mate:817, Mate:818, Mate:819, Mate:821, Mate:822
166. WireGuideToMiniSubExtender:1 — Mate:820, Mate:821, Mate:822
167. SmallSpoolAssembly:1 [sub-assembly] — Mate:826, Mate:827, Flush:120
168. CarriageImproved:1 — Mate:828, Mate:829, Mate:850, Mate:851, Mate:852, Mate:853, Mate:854, Mate:855, Angle:58, Mate:856, Mate:857, Angle:59
169. SleeveBearing.125inch:8 — Mate:830, Mate:831, Mate:1033
170. MiniSpoolServoShaft:1 — Mate:836, Mate:841, Mate:1033, Mate:1034
171. SleeveBearing.125inch:9 — Mate:837, Mate:838
172. ORingA50_.25OD_.125ID:70 — Rigid:28
173. ORingA50_.25OD_.125ID:71 — Rigid:31
174. CarriageConnectorShaft:1 — Mate:839, Mate:843, Mate:867, Flush:505
175. SleeveBearing.125inch:10 — Mate:840, Flush:122
176. largeIdlerPinion:4 — Mate:843, Flush:504, Mate:1114, Mate:1115, Mate:1116
177. smallIdlerPinion:7 — Mate:841, Mate:1105, Flush:504
178. carriageRideShaft:1 — Mate:845, Mate:846
179. spoolCarriageThreadedRodThread_5_40:1 — Mate:847, Mate:848, Mate:864, Mate:880
180. bearing_1_8inch:14 — Mate:849, Flush:124
181. SleeveBearing.125inch:11 — Mate:850, Mate:851
182. SleeveBearing.125inch:12 — Mate:852, Mate:853
183. NarrowHexNutThread_5_40:173 — Mate:856, Mate:857, Angle:59
184. NarrowHexNutThread_5_40:174 — Mate:854, Mate:855, Angle:58
185. PinionGear20T:1 — Mate:864, Mate:865, Flush:129
186. SleeveBearing.125inch:13 — Mate:866, Flush:127
187. smallIdlerPinion:8 — Mate:867, Flush:129, Flush:505
188. CarrageRodEndMount:1 — Mate:876, Mate:877, Mate:878, Mate:879, Mate:880, Mate:882, Mate:884, Mate:885, Mate:888
189. bearing_1_8inch:15 — Mate:878, Mate:879
190. NarrowHexNutThread_5_40:187 — Mate:881, Mate:882
191. NarrowHexNutThread_5_40:188 — Mate:883, Mate:884
192. NarrowHexNutThread_5_40:189 — Mate:885, Mate:886
193. NarrowHexNutThread_5_40:190 — Mate:887, Mate:888
194. SpoolServoMount:1 — Mate:890, Mate:891, Mate:892, Mate:898, Mate:900, Mate:906, Mate:908
195. ScrewPlastic_4_20_.5inch:32 — Mate:893, Mate:894
196. ScrewPlastic_4_20_.5inch:33 — Mate:895, Mate:896
197. NarrowHexNutThread_5_40:191 — Mate:897, Mate:898
198. NarrowHexNutThread_5_40:192 — Mate:899, Mate:900
199. NarrowHexNutThread_5_40:196 — Mate:905, Mate:906
200. NarrowHexNutThread_5_40:197 — Mate:907, Mate:908
201. ORingA70_2.484ID_2.762OD_Compressed:1 — Rigid:33
202. SleeveBearing.125inch:15 — Mate:914, Flush:132
203. ORingA50_.25OD_.125ID:78 — Rigid:34
204. 4mmShaftCollar:1 — Mate:921, Mate:929, Mate:930
205. ShaftCollarMagnetMount:1 — Mate:929, Mate:930, Mate:931, Flush:138, Mate:932, Flush:139
206. EncoderMagnet:1 — Mate:932, Flush:139
207. EncoderMagnet:2 — Mate:931, Flush:138
208. bearing_1_8inch:16 — Mate:979, Mate:1095, Mate:1096
209. bearing_1_8inch:17 — Mate:981, Mate:1091, Mate:1092
210. bearing_1_8inch:18 — Mate:983, Mate:1088, Mate:1089
211. bearing_1_8inch:19 — Mate:965, Flush:146
212. bearing_1_8inch:20 — Mate:966, Flush:147
213. bearing_1_8inch:21 — Mate:967, Flush:148
214. 540DCMotor:1 — Mate:971, Mate:972, Mate:973, Mate:977, Mate:978
215. BearingRetentionBrace:1 — Mate:974, Mate:975, Mate:976, Mate:997, Flush:154, Mate:998, Flush:155
216. idlerShaftBearingMount:1 — Mate:968, Mate:969, Mate:970, Mate:971, Mate:972, Mate:973
217. idlerShaft:1 — Mate:979, Mate:985, Mate:986, Rotation:4, Rotation:5, Mate:1097
218. smallIdlerPinion:9 — Mate:977, Mate:978, Flush:150, Rotation:3
219. idlerShaft2:1 — Mate:981, Mate:987, Mate:988, Rotation:6, Rotation:7, Mate:1093
220. idlerShaft2:2 — Mate:983, Mate:989, Mate:990, Rotation:8, Rotation:9, Mate:1090
221. largeIdlerPinion:5 — Mate:985, Flush:150, Rotation:3, Rotation:4
222. largeIdlerPinion:6 — Mate:987, Flush:151, Rotation:2, Rotation:7, Mate:1094
223. largeIdlerPinion:7 — Mate:989, Flush:152, Mate:993, Rotation:1, Rotation:8
224. smallIdlerPinion:10 — Mate:986, Flush:151, Rotation:2, Rotation:5
225. smallIdlerPinion:11 — Mate:988, Flush:152, Mate:992, Rotation:1, Rotation:6
226. smallIdlerPinion:12 — Mate:990, Mate:993, Rotation:9, Rotation:10
227. NarrowHexNutThread_5_40:201 — Mate:994, Mate:995
228. flatPlasticScrewSmall:64 — Mate:997, Flush:154
229. flatPlasticScrewSmall:65 — Mate:998, Flush:155
230. Bolt_SocketHead_Hex_Thread_M3_16mm:1 — Mate:999, Mate:1000
231. Bolt_SocketHead_Hex_Thread_M3_16mm:2 — Mate:1001, Mate:1002
232. pistonSpurGear:1 — Mate:1005, Mate:1006, Mate:1012, Angle:64, Mate:1013, Angle:65, Rotation:10, Rotation/Translation:1
233. CompressionWasherPlastic:1 — Mate:1007, Mate:1008, Angle:63
234. ThrustWasherPrimary:1 — Mate:1014, Mate:1015, Mate:1028
235. smallIdlerPinion:13 — Mate:1022, Mate:1024, Mate:1026
236. pushSwitchRodSpacer:1 — Mate:1025, Mate:1026
237. ThrustWasherPrimary:2 — Mate:1027, Mate:1028
238. ScimitarPropellerModel1:1 [sub-assembly] — Mate:1029, Mate:1030
239. 3mm_.125inch_ShaftCoupler:1 — Mate:1034, Mate:1040, Mate:1041, Angle:68, Mate:1105
240. GearMotorMount:1 — Mate:1037, Mate:1039, Angle:67, Mate:1041, Mate:1043, Mate:1045, Mate:1047, Mate:1104, Flush:501
241. MicroGearMotor:1 — Mate:1039, Mate:1040, Angle:67, Angle:69
242. NarrowHexNutThread_5_40:202 — Mate:1042, Mate:1043
243. NarrowHexNutThread_5_40:203 — Mate:1044, Mate:1045, Angle:69
244. NarrowHexNutThread_5_40:204 — Mate:1046, Mate:1047
245. NarrowHexNutThread_5_40:205 — Mate:1048, Mate:1049
246. ASDSAttachmentAssemblyUpdated:1 [sub-assembly] — Mate:1059, Angle:71, Flush:492, Flush:493
247. RearMount:1 — Mate:1060, Flush:492, Flush:493
248. hallEffectSensorAssembly:1 [sub-assembly] — Mate:1061, Mate:1062, Mate:1063, Flush:494, Flush:495
249. flatPlasticScrewSmall:66 — Mate:1064, Flush:494
250. flatPlasticScrewSmall:67 — Mate:1065, Flush:495
251. gearboxBearingHolderForward:1 — Mate:1072, Mate:1073, Mate:1074, Mate:1084, Mate:1085, Mate:1086, Mate:1087, Mate:1088, Mate:1091, Mate:1094, Mate:1095
252. gearboxBearingHolderHexNutBacking:1 — Mate:1075, Mate:1076, Mate:1077, Mate:1078, Mate:1079, Mate:1080, Mate:1081, Angle:74, Mate:1082, Mate:1083, Angle:75
253. flatPlasticScrewSmall:68 — Mate:1078, Flush:499
254. flatPlasticScrewSmall:69 — Mate:1079, Flush:500
255. HexNutThread_M3:4 — Mate:1080, Mate:1081, Angle:74
256. HexNutThread_M3:5 — Mate:1082, Mate:1083, Angle:75
257. Bolt_SocketHead_Hex_Thread_M3_8mm:1 — Mate:1084, Mate:1085, Angle:77
258. Bolt_SocketHead_Hex_Thread_M3_8mm:2 — Mate:1086, Mate:1087, Angle:76
259. GearMotorMountArm:1 — Mate:1103, Mate:1104, Flush:501, Mate:1049
260. NarrowHexNutThread_5_40:209 — Mate:1106, Angle:78, Mate:1108
261. NarrowHexNutThread_5_40:210 — Mate:1107, Angle:78, Angle:79, Mate:1110
262. HallEffectSpoolSensorMount2:1 — Mate:1108, Flush:502, Mate:1110, Angle:80, Mate:1111, Flush:503, Mate:1112, Mate:1113
263. HallEffectSensor:1 — Mate:1111, Flush:503, Mate:1112
264. SpoolCarrageMagnetMountREV2:1 — Mate:1115, Mate:1116, Mate:1117, Mate:1118
265. HallEffectSpoolSensorMount3:1 — Mate:1122, Mate:1123, Mate:1130, Angle:83, Mate:1133, Mate:1134, Flush:506
266. HallEffectSpoolSensorMount3Brace:1 — Mate:1120, Mate:1121, Mate:1122, Mate:1123, Mate:1125, Mate:1127, Mate:1128, Mate:1129, Mate:1132
267. NarrowHexNutThread_5_40:211 — Mate:1124, Mate:1125, Angle:81, Angle:82
268. NarrowHexNutThread_5_40:212 — Mate:1126, Mate:1127, Angle:81
269. Bolt_ButtonHead_Hex_Thread_M3_10mm:4 — Mate:1129, Mate:1130, Angle:83, Mate:1131
270. HexNutThread_M3:6 — Mate:1131, Mate:1132, Angle:84
271. HallEffectSensor:2 — Mate:1133, Mate:1134, Flush:506
272. HallEffectSpoolSensorMount3:2 — Mate:1135, Mate:1136, Mate:1137, Mate:1138, Angle:87
273. ScrewPlastic_4_20_.5inch:38 — Mate:1137, Mate:1138
274. NarrowHexNutThread_5_40:213 — Mate:1139, Mate:1140, Angle:88
275. NarrowHexNutThread_5_40:214 — Mate:1141, Mate:1142, Angle:89
276. RelayHolderREV2:1 — Mate:1143, Mate:1144, Mate:1145, Mate:1146, Angle:90
277. SlipRingAssy:1 [sub-assembly] — Mate:1147, Mate:1148
278. Bolt_ButtonHead_Hex_Thread_5_40_1inch:1 — Mate:206, Mate:216
279. Bolt_ButtonHead_Hex_Thread_5_40_1inch:2 — Mate:307
280. Bolt_ButtonHead_Hex_Thread_5_40_1inch:3
281. Bolt_ButtonHead_Hex_Thread_5_40_1inch:4
282. NarrowHexNutThread_5_40:5 — Mate:205, Angle:13, Mate:437, Flush:491
283. NarrowHexNutThread_5_40:6
284. NarrowHexNutThread_5_40:7
285. NarrowHexNutThread_5_40:8
286. NarrowHexNutThread_5_40:9
287. NarrowHexNutThread_5_40:10
288. NarrowHexNutThread_5_40:3 — Mate:190, Angle:11, Mate:307
289. NarrowHexNutThread_5_40:11
290. NarrowHexNutThread_5_40:12
291. NarrowHexNutThread_5_40:13
292. NarrowHexNutThread_5_40:14 — Mate:219, Mate:220, Angle:14
293. NarrowHexNutThread_5_40:15
294. NarrowHexNutThread_5_40:16
295. NarrowHexNutThread_5_40:17
296. NarrowHexNutThread_5_40:18
297. NarrowHexNutThread_5_40:19 — Flush:125
298. ORingA50_.25OD_.125ID:24 — Rigid:11
299. ORingA50_.25OD_.125ID:25
300. ORingA50_.25OD_.125ID:26
301. ORingA50_.25OD_.125ID:27
302. Bolt_Buttonhead_Hex_Thread_5_40_.625inch:1 — Mate:228, Mate:229, Mate:230
303. Bolt_Buttonhead_Hex_Thread_5_40_.625inch:2
304. Bolt_Buttonhead_Hex_Thread_5_40_.625inch:3
305. Bolt_Buttonhead_Hex_Thread_5_40_.625inch:4
306. NarrowHexNutThread_5_40:20 — Mate:230, Mate:231, Angle:17
307. NarrowHexNutThread_5_40:21
308. NarrowHexNutThread_5_40:22
309. NarrowHexNutThread_5_40:23
310. ScrewPlastic_4_20_.75inch_Flat:1 — Mate:244, Flush:18
311. ScrewPlastic_4_20_.75inch_Flat:2
312. ScrewPlastic_4_20_.75inch_Flat:3
313. ScrewPlastic_4_20_.75inch_Flat:4
314. ScrewPlastic_4_20_.75inch_Flat:5
315. ScrewPlastic_4_20_.75inch_Flat:6
316. NarrowHexNutThread_5_40:24 — Mate:249, Mate:275, Angle:70
317. NarrowHexNutThread_5_40:25
318. NarrowHexNutThread_5_40:26
319. NarrowHexNutThread_5_40:27
320. NarrowHexNutThread_5_40:28
321. NarrowHexNutThread_5_40:29
322. ORingA50_.25OD_.125ID:34 — Rigid:35
323. ORingA50_.25OD_.125ID:35
324. ORingA50_.25OD_.125ID:36
325. ORingA50_.25OD_.125ID:37
326. ORingA50_.25OD_.125ID:38
327. ORingA50_.25OD_.125ID:39
328. NarrowHexNutThread_5_40:50 — Mate:301, Mate:302, Mate:303, Flush:25
329. NarrowHexNutThread_5_40:51
330. NarrowHexNutThread_5_40:52
331. NarrowHexNutThread_5_40:53
332. NarrowHexNutThread_5_40:54
333. NarrowHexNutThread_5_40:55
334. aftThreadedRodThread_5_40:1 — Mate:303, Flush:25, Mate:304, Mate:422, Mate:876, Mate:881, Mate:883
335. aftThreadedRodThread_5_40:2 — Mate:374, Mate:420, Mate:425, Mate:460, Mate:877, Mate:886, Mate:887, Flush:149
336. aftThreadedRodThread_5_40:3
337. aftThreadedRodThread_5_40:4
338. aftThreadedRodThread_5_40:5
339. aftThreadedRodThread_5_40:6 — Mate:386
340. NarrowHexNutThread_5_40:56 — Mate:304, Mate:305
341. NarrowHexNutThread_5_40:57
342. NarrowHexNutThread_5_40:58
343. NarrowHexNutThread_5_40:59
344. NarrowHexNutThread_5_40:60
345. NarrowHexNutThread_5_40:61
346. ScrewPlastic_4_20_.75inch_Flat:19 — Mate:385, Flush:52
347. ScrewPlastic_4_20_.75inch_Flat:20
348. ScrewPlastic_4_20_.75inch_Flat:21
349. ScrewPlastic_4_20_.75inch_Flat:22
350. ScrewPlastic_4_20_.75inch_Flat:23
351. ScrewPlastic_4_20_.75inch_Flat:24
352. NarrowHexNutThread_5_40:66 — Mate:386, Mate:387
353. NarrowHexNutThread_5_40:67
354. NarrowHexNutThread_5_40:68
355. NarrowHexNutThread_5_40:69
356. NarrowHexNutThread_5_40:70
357. NarrowHexNutThread_5_40:71
358. ScrewPlastic_4_20_.5inch:18 — Mate:412, Mate:413
359. ScrewPlastic_4_20_.5inch:19
360. ScrewPlastic_4_20_.5inch:20
361. ORingA50_.25OD_.125ID:40 — Rigid:20
362. ORingA50_.25OD_.125ID:41
363. ORingA50_.25OD_.125ID:42
364. ORingA50_.25OD_.125ID:43
365. ORingA50_.25OD_.125ID:44
366. ORingA50_.25OD_.125ID:45
367. Bolt_Buttonhead_Hex_Thread_5_40_.625inch:5 — Mate:414, Mate:415, Mate:416
368. Bolt_Buttonhead_Hex_Thread_5_40_.625inch:6
369. Bolt_Buttonhead_Hex_Thread_5_40_.625inch:7
370. Bolt_Buttonhead_Hex_Thread_5_40_.625inch:8
371. Bolt_Buttonhead_Hex_Thread_5_40_.625inch:9
372. Bolt_Buttonhead_Hex_Thread_5_40_.625inch:10
373. NarrowHexNutThread_5_40:72 — Mate:416, Mate:417
374. NarrowHexNutThread_5_40:73
375. NarrowHexNutThread_5_40:74
376. NarrowHexNutThread_5_40:75
377. NarrowHexNutThread_5_40:76
378. NarrowHexNutThread_5_40:77
379. ORingA50_.25OD_.125ID:46 — Rigid:37
380. ORingA50_.25OD_.125ID:47
381. ORingA50_.25OD_.125ID:48
382. ORingA50_.25OD_.125ID:49
383. ORingA50_.25OD_.125ID:50
384. ORingA50_.25OD_.125ID:51
385. NarrowHexNutThread_5_40:84 — Mate:444, Mate:445, Angle:28
386. NarrowHexNutThread_5_40:85
387. NarrowHexNutThread_5_40:86
388. NarrowHexNutThread_5_40:87
389. NarrowHexNutThread_5_40:88
390. NarrowHexNutThread_5_40:89
391. midshipsThreadedRodThread_5_40:1 — Mate:446, Mate:1021, Angle:36, Mate:644, Mate:646, Mate:665, Mate:666, Mate:780, Mate:1141, Mate:1143
392. midshipsThreadedRodThread_5_40:2 — Mate:485, Mate:586, Mate:589, Mate:592, Flush:91, Mate:593, Mate:595, Mate:645, Mate:655, Mate:662, Mate:694, Tangent:5, Mate:994
393. midshipsThreadedRodThread_5_40:3 — Mate:647, Mate:688, Mate:690, Mate:692, Tangent:6, Mate:726
394. midshipsThreadedRodThread_5_40:4 — Mate:727
395. midshipsThreadedRodThread_5_40:5
396. midshipsThreadedRodThread_5_40:6 — Mate:475, Mate:657, Mate:664, Mate:667, Mate:673, Mate:675, Mate:681, Mate:1139, Mate:1144
397. NarrowHexNutThread_5_40:90 — Mate:460, Mate:461, Angle:73
398. NarrowHexNutThread_5_40:91
399. NarrowHexNutThread_5_40:92
400. NarrowHexNutThread_5_40:93
401. NarrowHexNutThread_5_40:94
402. NarrowHexNutThread_5_40:95
403. flatPlasticScrewSmall:21 — Mate:466, Flush:61
404. flatPlasticScrewSmall:22
405. flatPlasticScrewSmall:23
406. flatPlasticScrewSmall:24
407. retentionStandoffs:1 — Mate:475, Mate:476, Angle:32
408. retentionStandoffs:2 — Mate:480
409. retentionStandoffs:3 — Mate:482
410. retentionStandoffs:4
411. retentionStandoffs:5
412. retentionStandoffs:6
413. NarrowHexNutThread_5_40:99 — Mate:485, Mate:486
414. NarrowHexNutThread_5_40:100
415. NarrowHexNutThread_5_40:101
416. NarrowHexNutThread_5_40:102
417. NarrowHexNutThread_5_40:103
418. NarrowHexNutThread_5_40:104
419. flatPlasticScrewSmall:36 — Mate:526, Flush:74
420. flatPlasticScrewSmall:37
421. flatPlasticScrewSmall:38
422. ORingA50_.25OD_.125ID:52 — Rigid:24
423. ORingA50_.25OD_.125ID:53
424. ORingA50_.25OD_.125ID:54
425. ORingA50_.25OD_.125ID:55
426. ORingA50_.25OD_.125ID:56
427. ORingA50_.25OD_.125ID:57
428. NarrowHexNutThread_5_40:105 — Mate:593, Mate:594
429. NarrowHexNutThread_5_40:106
430. NarrowHexNutThread_5_40:107
431. NarrowHexNutThread_5_40:108
432. NarrowHexNutThread_5_40:109
433. NarrowHexNutThread_5_40:110 — Mate:915, Mate:916, Mate:917
434. NarrowHexNutThread_5_40:111 — Mate:595, Mate:596
435. NarrowHexNutThread_5_40:112
436. NarrowHexNutThread_5_40:113
437. NarrowHexNutThread_5_40:114
438. NarrowHexNutThread_5_40:115
439. NarrowHexNutThread_5_40:116
440. ScrewPlastic_4_20_.5inch:25 — Mate:599, Mate:600
441. ScrewPlastic_4_20_.5inch:26
442. ScrewPlastic_4_20_.5inch:27
443. ScrewPlastic_4_20_.5inch:28
444. NarrowHexNutThread_5_40:117 — Mate:631, Mate:632, Angle:42
445. NarrowHexNutThread_5_40:118
446. NarrowHexNutThread_5_40:119
447. NarrowHexNutThread_5_40:120
448. NarrowHexNutThread_5_40:121
449. NarrowHexNutThread_5_40:122
450. Bolt_Buttonhead_Hex_Thread_5_40_.625inch:11 — Mate:636, Mate:637
451. Bolt_Buttonhead_Hex_Thread_5_40_.625inch:12
452. Bolt_Buttonhead_Hex_Thread_5_40_.625inch:13
453. Bolt_Buttonhead_Hex_Thread_5_40_.625inch:14
454. Bolt_Buttonhead_Hex_Thread_5_40_.625inch:15
455. Bolt_Buttonhead_Hex_Thread_5_40_.625inch:16
456. flatPlasticScrewSmall:54 — Mate:643, Flush:104
457. flatPlasticScrewSmall:55
458. flatPlasticScrewSmall:56
459. flatPlasticScrewSmall:57
460. flatPlasticScrewSmall:58
461. flatPlasticScrewSmall:59
462. NarrowHexNutThread_5_40:135 — Mate:662, Mate:663
463. NarrowHexNutThread_5_40:136
464. NarrowHexNutThread_5_40:137
465. NarrowHexNutThread_5_40:159 — Mate:688, Mate:689
466. NarrowHexNutThread_5_40:160
467. NarrowHexNutThread_5_40:161
468. NarrowHexNutThread_5_40:165 — Mate:690, Mate:691
469. NarrowHexNutThread_5_40:166
470. NarrowHexNutThread_5_40:167
471. aftServoSectionThreadedRodThread_5_40:1 — Mate:858, Flush:125, Mate:859, Mate:861, Flush:126, Angle:66, Mate:1046, Mate:1048, Mate:1103
472. NarrowHexNutThread_5_40:175 — Mate:859, Mate:860
473. ORingA50_.25OD_.125ID:72 — Rigid:36
474. NarrowHexNutThread_5_40:176 — Mate:861, Flush:126
475. aftServoSectionThreadedRodThread_5_40:2 — Mate:890, Mate:905, Mate:907, Mate:1106, Mate:1107, Mate:1113
476. NarrowHexNutThread_5_40:177
477. ORingA50_.25OD_.125ID:73
478. NarrowHexNutThread_5_40:178
479. aftServoSectionThreadedRodThread_5_40:3
480. NarrowHexNutThread_5_40:179
481. ORingA50_.25OD_.125ID:74
482. NarrowHexNutThread_5_40:180
483. aftServoSectionThreadedRodThread_5_40:4 — Mate:891, Mate:897, Mate:899
484. NarrowHexNutThread_5_40:181
485. ORingA50_.25OD_.125ID:75
486. NarrowHexNutThread_5_40:182
487. aftServoSectionThreadedRodThread_5_40:5 — Mate:1121, Mate:1124, Mate:1126
488. NarrowHexNutThread_5_40:183
489. ORingA50_.25OD_.125ID:76
490. NarrowHexNutThread_5_40:184
491. aftServoSectionThreadedRodThread_5_40:6 — Mate:1037, Mate:1042, Mate:1044, Mate:1120
492. NarrowHexNutThread_5_40:185
493. ORingA50_.25OD_.125ID:77
494. NarrowHexNutThread_5_40:186
495. NarrowHexNutCaps:1 — Mate:915, Mate:916, Mate:917
496. NarrowHexNutCaps:2
497. NarrowHexNutCaps:3
498. NarrowHexNutCaps:4
499. NarrowHexNutCaps:5
500. NarrowHexNutCaps:6
501. ScrewPlastic_4_20_.5inch:34 — Mate:1003, Mate:1004
502. ScrewPlastic_4_20_.5inch:35
503. ScrewPlastic_4_20_.5inch:36
504. ScrewPlastic_4_20_.5inch:37
505. HexNutThread_M3:1 — Mate:1012, Mate:1102
506. HexNutThread_M3:2
507. HexNutThread_M3:3
508. ORingA50_.25OD_.125ID:79 — Rigid:38
509. Bolt_ButtonHead_Hex_Thread_5_40_1inch:5 — Mate:1031, Flush:491
510. ORingA50_.25OD_.125ID:80 — Rigid:39
511. ORingA50_.25OD_.125ID:81
512. Bolt_ButtonHead_Hex_Thread_5_40_1inch:6
513. ORingA50_.25OD_.125ID:82
514. ORingA50_.25OD_.125ID:83
515. Bolt_ButtonHead_Hex_Thread_5_40_1inch:7
516. ORingA50_.25OD_.125ID:84
517. ORingA50_.25OD_.125ID:85
518. Bolt_ButtonHead_Hex_Thread_5_40_1inch:8
519. ORingA50_.25OD_.125ID:86
520. ORingA50_.25OD_.125ID:87
521. Bolt_ButtonHead_Hex_Thread_5_40_1inch:9
522. ORingA50_.25OD_.125ID:88
523. ORingA50_.25OD_.125ID:89
524. Bolt_ButtonHead_Hex_Thread_5_40_1inch:10
525. ORingA50_.25OD_.125ID:90
526. Bolt_ButtonHead_Hex_Thread_M3_10mm:1 — Mate:1100, Mate:1101
527. Bolt_ButtonHead_Hex_Thread_M3_10mm:2
528. Bolt_ButtonHead_Hex_Thread_M3_10mm:3 — Mate:1102
529. EncoderMagnet:3 — Mate:1117, Mate:1118
530. EncoderMagnet:4
531. EncoderMagnet:5
532. EncoderMagnet:6
533. RelayModule:1 — Mate:1145, Mate:1146, Angle:90
534. RelayModule:2
535. ScrewPlastic_4_20_.5inch:2 — Mate:296, Mate:297
536. ScrewPlastic_4_20_.5inch:3
537. ScrewPlastic_4_20_.5inch:4
538. ScrewPlastic_4_20_.5inch:5
539. ScrewPlastic_4_20_.5inch:6
540. ScrewPlastic_4_20_.5inch:7
541. ScrewPlastic_4_20_.5inch:8
542. ScrewPlastic_4_20_.5inch:9
543. ORingA70_.176ID_.316OD:1 — Rigid:17
544. ORingA70_.176ID_.316OD:2
545. ORingA70_.176ID_.316OD:3
546. ORingA70_.176ID_.316OD:4
547. ORingA70_.176ID_.316OD:5
548. ORingA70_.176ID_.316OD:6
549. aluminumWiringTubing:1 — Mate:300, Flush:153
550. aluminumWiringTubing:2
551. aluminumWiringTubing:3
552. aluminumWiringTubing:4
553. aluminumWiringTubing:5
554. aluminumWiringTubing:6
555. ORingA70_.176ID_.316OD:7 — Rigid:23
556. ORingA70_.176ID_.316OD:8
557. ORingA70_.176ID_.316OD:9
558. ORingA70_.176ID_.316OD:10
559. ORingA70_.176ID_.316OD:11